# Autodesk Inventor assembly: Actuador Cremallera
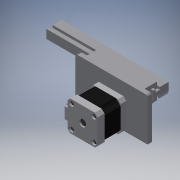
[picture p0: Inventor's stored thumbnail of the model, 180x180]
Saved by Autodesk Inventor 2019 (Build 230136000, 136)
## iProperties
Created: 2020-02-02
Part Number: Actuador Cremallera
Document SubType Name: Assembly
Designer: Elías Sánchez
Author: Elías Sánchez
## Documents named in this file (11)
- D:\Documents\UVG\9no SEMESTRE\DISEÑO E INNOVACIÓN\Proyecto Actuadores\Inventor Actuadores\Actuador Cremallera\Actuador Cremallera.iam
- D:\Documents\UVG\9no SEMESTRE\DISEÑO E INNOVACIÓN\Proyecto Actuadores\Inventor Actuadores\Actuador Cremallera\Acople eje motor.ipt
- D:\Documents\UVG\9no SEMESTRE\DISEÑO E INNOVACIÓN\Proyecto Actuadores\Inventor Actuadores\Actuador Cremallera\Engrane\Design Accelerator\Spur Gear11.ipt
- D:\Documents\UVG\9no SEMESTRE\DISEÑO E INNOVACIÓN\Proyecto Actuadores\Inventor Actuadores\Actuador Cremallera\Cremallera.ipt
- D:\Documents\UVG\9no SEMESTRE\DISEÑO E INNOVACIÓN\Proyecto Actuadores\Inventor Actuadores\Actuador Cremallera\Riel cremallera p1.ipt
- D:\Documents\UVG\9no SEMESTRE\DISEÑO E INNOVACIÓN\Proyecto Actuadores\Inventor Actuadores\Actuador Cremallera\Riel cremallera p2.ipt
- D:\Documents\UVG\9no SEMESTRE\DISEÑO E INNOVACIÓN\Proyecto Actuadores\Inventor Actuadores\Actuador Cremallera\Nema 17\Nema_17-17HS4401.iam
- D:\Documents\UVG\9no SEMESTRE\DISEÑO E INNOVACIÓN\Proyecto Actuadores\Inventor Actuadores\Actuador Cremallera\Tope riel motor.ipt
- D:\Documents\UVG\9no SEMESTRE\DISEÑO E INNOVACIÓN\Proyecto Actuadores\Inventor Actuadores\Actuador Cremallera\Riel acople de motor.ipt
- D:\Documents\UVG\9no SEMESTRE\DISEÑO E INNOVACIÓN\Proyecto Actuadores\Inventor Actuadores\Actuador Cremallera\M3.5.ipt
- D:\Documents\UVG\9no SEMESTRE\DISEÑO E INNOVACIÓN\Proyecto Actuadores\Inventor Actuadores\Actuador Cremallera\M3.ipt
## Components (13 placed, 10 different names)
1. Acople eje motor:1 — Mate:1, Mate:2, Angle:1, Mate:4, Insert:6
2. Engrane:1 — Mate:1, Mate:2, Angle:1, Mate:3, Flush:7, Mate:7, Rotation/Translation:1
3. Cremallera:1 — Mate:5, Flush:1, Flush:2, Flush:5, Flush:6, Flush:7, Mate:7, Rotation/Translation:1, Flush:10
4. Riel cremallera p1:1 — Mate:5, Flush:1, Flush:2, Mate:6, Flush:3, Flush:4, Flush:11
5. Riel cremallera p2:1 — Mate:6, Flush:3, Flush:4
6. Nema_17-17HS4401:1 [sub-assembly] — Mate:3, Mate:4, Angle:2, Insert:1, Flush:8
7. Tope riel motor:1 — Insert:1, Flush:8, Mate:8, Mate:9, Flush:9, Insert:2, Insert:3, Insert:4, Insert:5
8. Riel acople de motor:1 — Mate:8, Mate:9, Flush:9, Flush:10, Flush:11
9. M3.5:1 — Insert:5
10. M3.5:2 — Insert:2
11. M3.5:3 — Insert:3
12. M3.5:4 — Insert:4
13. M3:1 — Insert:6
## Relationships (29: Flush 11, Mate 9, Insert 6, Angle 2, RelateRotateTranslate 1)
- Mate:1: Acople eje motor:1 ↔ Engrane:1
- Mate:2: Acople eje motor:1 ↔ Engrane:1
- Angle:1 (0 deg): Acople eje motor:1 ↔ Engrane:1
- Mate:3: Engrane:1 ↔ Nema_17-17HS4401:1
- Mate:4: Acople eje motor:1 ↔ Nema_17-17HS4401:1
- Mate:5: Cremallera:1 ↔ Riel cremallera p1:1
- Flush:1: Cremallera:1 ↔ Riel cremallera p1:1
- Flush:2 (3.5 mm): Cremallera:1 ↔ Riel cremallera p1:1
- Mate:6: Riel cremallera p1:1 ↔ Riel cremallera p2:1
- Flush:3: Riel cremallera p1:1 ↔ Riel cremallera p2:1
- Flush:4 (-3.5 mm): Riel cremallera p1:1 ↔ Riel cremallera p2:1
- Flush:5: Cremallera:1
- Flush:6: Cremallera:1
- Flush:7: Engrane:1 ↔ Cremallera:1
- Angle:2 (0 deg): Nema_17-17HS4401:1
- Mate:7 (23 mm): Engrane:1 ↔ Cremallera:1
- Rotation/Translation:1 [RelateRotateTranslate] (-125.5 mm): Engrane:1 ↔ Cremallera:1
- Insert:1 (-4.5 mm): Nema_17-17HS4401:1 ↔ Tope riel motor:1
- Flush:8: Nema_17-17HS4401:1 ↔ Tope riel motor:1
- Mate:8: Tope riel motor:1 ↔ Riel acople de motor:1
- Mate:9: Tope riel motor:1 ↔ Riel acople de motor:1
- Flush:9: Tope riel motor:1 ↔ Riel acople de motor:1
- Flush:10: Cremallera:1 ↔ Riel acople de motor:1
- Flush:11: Riel cremallera p1:1 ↔ Riel acople de motor:1
- Insert:2: Tope riel motor:1 ↔ M3.5:2
- Insert:3: Tope riel motor:1 ↔ M3.5:3
- Insert:4: Tope riel motor:1 ↔ M3.5:4
- Insert:5: Tope riel motor:1 ↔ M3.5:1
- Insert:6: Acople eje motor:1 ↔ M3:1
